# Autodesk Inventor assembly: 30 full stop
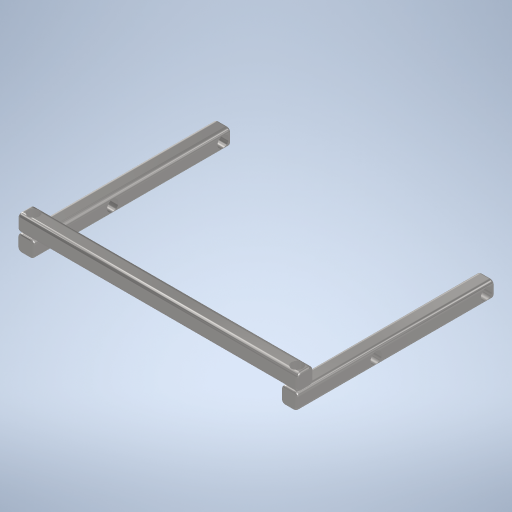
[picture p0: Inventor's stored thumbnail of the model, 512x512]
Saved by Autodesk Inventor 2023 (Build 270158000, 158)
## iProperties
Created: 2022-09-27
Part Number: 30 full stop
Document SubType Name: Assembly
Designer: aaron
Author: aaron
## Documents named in this file (3)
- C:\Users\aaron\Documents\Inventor\Spin Up\library\Structure\hs shaft\30 full stop.iam
- C:\Users\aaron\Documents\Inventor\Spin Up\library\Structure\hs shaft\30 stop.ipt
- C:\Users\aaron\Documents\Inventor\Spin Up\library\Structure\hs shaft\beam.ipt
## Components (3 placed, 2 different names)
1. 30 stop:1 — Mate:1, Mate:2, Flush:1, Flush:2, Mate:6, Mate:7
2. beam:1 — Mate:1, Flush:1, Mate:5, Mate:6
3. beam:2 — Mate:2, Flush:2, Mate:5, Mate:7
## Relationships (7: Mate 5, Flush 2)
- Mate:1: 30 stop:1 ↔ beam:1
- Mate:2: 30 stop:1 ↔ beam:2
- Flush:1: 30 stop:1 ↔ beam:1
- Flush:2: 30 stop:1 ↔ beam:2
- Mate:5: beam:1 ↔ beam:2
- Mate:6: 30 stop:1 ↔ beam:1
- Mate:7: 30 stop:1 ↔ beam:2
